# Autodesk Inventor assembly: Small-Servo-Holder
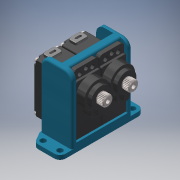
[picture p0: Inventor's stored thumbnail of the model, 180x180]
Saved by Autodesk Inventor 2018.2 (Build 222227000, 227)
## iProperties
Created: 2018-02-21
Part Number: Small-Servo-Holder
Material: Generisch
Document SubType Name: Assembly
Designer: JochenAlt
Author: JochenAlt
## Documents named in this file (3)
- D:\Projects\Donna\CAD\Servo-Holder-Small.iam
- D:\Projects\Donna\CAD\Stewart-Servo-Holder-Small.ipt
- D:\Projects\Donna\CAD\Hitec HS-5065MG.ipt
## Components (3 placed, 2 different names)
1. Stewart-Servo-Holder-Small:1 — Passend:1, Passend:2, Winkel:1, Winkel:2, Passend:3, Passend:4
2. Hitec HS-5065MG:1 — Passend:1, Winkel:1, Passend:3
3. Hitec HS-5065MG:2 — Passend:2, Winkel:2, Passend:4
## Relationships (6: Mate 4, Angle 2)
- Passend:1 [Mate]: Stewart-Servo-Holder-Small:1 ↔ Hitec HS-5065MG:1
- Passend:2 [Mate]: Stewart-Servo-Holder-Small:1 ↔ Hitec HS-5065MG:2
- Winkel:1 [Angle] (180 deg): Stewart-Servo-Holder-Small:1 ↔ Hitec HS-5065MG:1
- Winkel:2 [Angle] (180 deg): Stewart-Servo-Holder-Small:1 ↔ Hitec HS-5065MG:2
- Passend:3 [Mate]: Stewart-Servo-Holder-Small:1 ↔ Hitec HS-5065MG:1
- Passend:4 [Mate]: Stewart-Servo-Holder-Small:1 ↔ Hitec HS-5065MG:2
